# Autodesk Inventor assembly: HNTC5-5
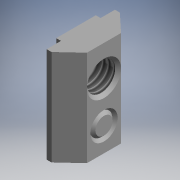
[picture p0: Inventor's stored thumbnail of the model, 180x180]
Saved by Autodesk Inventor 2017.3 (Build 213256000, 256)
## iProperties
Category: PARTsolutions
Company: MISUMI
Part Number: HNTC5-5
Catalog Web Link: www.cadenas.de
Description: HNTC5-Nuts for Aluminum Extrusions - Pre-Assembly Fitting Lock Nuts  - HFS5 Series (Aluminum Extrusions 20, 25, 40 Square)
Vendor: MISUMI
Document SubType Name: Assembly
Designer: partserver
Manufacturer: MISUMI
Mass: 0.387278 g
Surface Area: 5.33365 cm^2
Volume: 0.387278 cm^3
Density: 1 g/cm^3
Title: HNTC5-5
Author: Cadenas PARTsolutions
Comments: Nuts for Aluminum Extrusions - Pre-Assembly Fitting Lock Nuts  - HFS5 Series (Aluminum Extrusions 20, 25, 40 Square)
PSOL_IDENT_0: {$CADENAS_DATA\23d-libs\misumi\metric\38_al_extrusions_blackets\nuts\hntc5_asmtab.prj},167 {VTYP=3D}
PSOL_IDENT_1: ,{STYP=ASSTAB},{NB=HNTC5-5},{LINA=HNTC5-5},{NN=HNTC5},{DATE=28.07.2021 09:30:14},{GEOMDATE=13.02.201
PSOL_IDENT_2: 7 06:00:21},{VERSION=},{LINEID=10},{WBVAR=},{WBNUMERIC=}  {NB=HNTC5-5},{LINA=HNTC5-5},{KT=DUMMY},{PN=
PSOL_IDENT_3: HNTC5-5},{TYPE=HNTC5},{MAT=1010 Carbon Steel or Equivalent},{ST=Trivalent Chromate},{M=5},{AC=For Lo
PSOL_IDENT_4: ck M4 Set Screw (1pc.)},{RTT=6.8},{B=10.000},{L=14.000},{L1=3.500},{L2=4.500},{A=5.800},{E=3.400},{T=
PSOL_IDENT_5: 4.100},{W=5.000},{R1=0.000},{R2=0.000},{F=43.000},{LS=4.000},{PPATH=hntc5/hntc5_asmtpl.prj}
NB: HNTC5-5
NN: HNTC5
NT: Nuts for Aluminum Extrusions - Pre-Assembly Fitting Lock Nuts  - HFS5 Series (Aluminum Extrusions 20, 25, 40 Square)
NBSYN: $PN.
LINA: HNTC5-5
CATALOG: Misumi
PN: HNTC5-5
MAT: 1010 Carbon Steel or Equivalent
ST: Trivalent Chromate Plating
M: 5
AC: For Lock M4 Set Screw (1pc.)
RTT: 6.8
SUPPLIER: MISUMI
ARTICLENO: HNTC5-5
BOMINFO: HNTC5-5
CREATOR: CADENAS GmbH
## Documents named in this file (3)
- e:\temp\worker_41\temp\exporttempdir_4760_300_tQZoi\format_0\HNTC5-5.iam
- e:\temp\worker_41\temp\exporttempdir_4760_300_tQZoi\format_0\HNTC5_n.ipt
- e:\temp\worker_41\temp\exporttempdir_4760_300_tQZoi\format_0\Hexagon socket set screw with flat point DIN 913 - M4x4.ipt
## Components (2 placed, 2 different names)
1. HNTC5_n:1 — set_screw_Z@1 <-> IP2_Z@2
2. Hexagon socket set screw with flat point DIN 913 - M4x4:1 — set_screw_Z@1 <-> IP2_Z@2
## Relationships (1: Mate 1)
- set_screw_Z@1 <-> IP2_Z@2 [Mate]: HNTC5_n:1 ↔ Hexagon socket set screw with flat point DIN 913 - M4x4:1
